# Autodesk Inventor assembly: quadruped_bai_servo_assembly
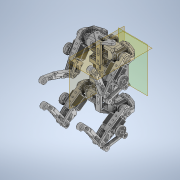
[picture p0: Inventor's stored thumbnail of the model, 180x180]
Saved by Autodesk Inventor 2022.1 (Build 261234020, 234B)
## iProperties
Created: 2022-02-06
Part Number: quadruped_bai_servo_assembly
Document SubType Name: Assembly
Designer: kee
Mass: 252.572 g
Surface Area: 1439.83 cm^2
Volume: 212.41 cm^3
Density: 1.18907 g/cm^3
Sending System: Autodesk Inventor 2020
Preprocessor: ST-DEVELOPER v18
Title: D:\open_source_projs\Quadruped_bai_servo\hardware\step\quadruped_bai_servo_assembly.stp
Author: Shuang Peng
## Documents named in this file (10)
- C:\Users\logic\_workspace\Quadruped_bai_servo\hardware\inventor\quadruped_bai_servo_assembly\quadruped_bai_servo_assembly.iam
- C:\Users\logic\_workspace\Quadruped_bai_servo\hardware\inventor\quadruped_bai_servo_assembly\leg_ass_1.iam
- C:\Users\logic\_workspace\Quadruped_bai_servo\hardware\inventor\quadruped_bai_servo_assembly\leg_ass_1_back.iam
- C:\Users\logic\_workspace\Quadruped_bai_servo\hardware\inventor\quadruped_bai_servo_assembly\leg_ass_1_MIR.iam
- C:\Users\logic\_workspace\Quadruped_bai_servo\hardware\inventor\quadruped_bai_servo_assembly\leg_ass_1_back_MIR.iam
- C:\Users\logic\_workspace\Quadruped_bai_servo\hardware\inventor\quadruped_bai_servo_assembly\body_frame_1.ipt
- C:\Users\logic\_workspace\Quadruped_bai_servo\hardware\inventor\quadruped_bai_servo_assembly\joint_ab_holder.ipt
- C:\Users\logic\_workspace\Quadruped_bai_servo\hardware\inventor\quadruped_bai_servo_assembly\body_frame_2.ipt
- C:\Users\logic\_workspace\Quadruped_bai_servo\hardware\inventor\quadruped_bai_servo_assembly\body_bridge_1.ipt
- C:\Users\logic\_workspace\Quadruped_bai_servo\hardware\inventor\quadruped_bai_servo_assembly\pcb_holder.ipt
## Components (12 placed, 9 different names)
1. leg_ass_1:1 [sub-assembly] — Insert:1, Insert:2
2. leg_ass_1_back:1 [sub-assembly] — Insert:5, Insert:6
3. leg_ass_1_MIR:1 [sub-assembly] — Insert:3, Insert:4
4. leg_ass_1_back_MIR:1 [sub-assembly] — Insert:7, Insert:8
5. body_frame_1:1 — Mate:1, Mate:2, Insert:1, Insert:2, Insert:3, Insert:4, Insert:5, Insert:6, Insert:7, Insert:8, Insert:17, Insert:18, Insert:19, Insert:20
6. joint_ab_holder:1 — Insert:15, Mate:4, Insert:20
7. joint_ab_holder:2 — Insert:14, Mate:3, Insert:19
8. body_frame_2:1 — Insert:9, Insert:10, Insert:11, Insert:12, Insert:13, Insert:16, Insert:17, Insert:18
9. body_bridge_1:1 — Insert:15, Mate:4, Insert:16
10. body_bridge_1:2 — Insert:13, Insert:14, Mate:3
11. pcb_holder:1 — Insert:9, Insert:10
12. pcb_holder:2 — Insert:11, Insert:12
## Relationships (24: Insert 20, Mate 4)
- Mate:1: body_frame_1:1
- Mate:2: body_frame_1:1
- Insert:1: leg_ass_1:1 ↔ body_frame_1:1
- Insert:2: leg_ass_1:1 ↔ body_frame_1:1
- Insert:3: leg_ass_1_MIR:1 ↔ body_frame_1:1
- Insert:4: leg_ass_1_MIR:1 ↔ body_frame_1:1
- Insert:5: leg_ass_1_back:1 ↔ body_frame_1:1
- Insert:6: leg_ass_1_back:1 ↔ body_frame_1:1
- Insert:7: leg_ass_1_back_MIR:1 ↔ body_frame_1:1
- Insert:8: leg_ass_1_back_MIR:1 ↔ body_frame_1:1
- Insert:9: body_frame_2:1 ↔ pcb_holder:1
- Insert:10: body_frame_2:1 ↔ pcb_holder:1
- Insert:11: body_frame_2:1 ↔ pcb_holder:2
- Insert:12: body_frame_2:1 ↔ pcb_holder:2
- Insert:13: body_frame_2:1 ↔ body_bridge_1:2
- Insert:14: joint_ab_holder:2 ↔ body_bridge_1:2
- Mate:3: joint_ab_holder:2 ↔ body_bridge_1:2
- Insert:15: joint_ab_holder:1 ↔ body_bridge_1:1
- Mate:4: joint_ab_holder:1 ↔ body_bridge_1:1
- Insert:16: body_frame_2:1 ↔ body_bridge_1:1
- Insert:17: body_frame_1:1 ↔ body_frame_2:1
- Insert:18: body_frame_1:1 ↔ body_frame_2:1
- Insert:19: body_frame_1:1 ↔ joint_ab_holder:2
- Insert:20: body_frame_1:1 ↔ joint_ab_holder:1
